# Autodesk Inventor assembly: 000-A-000
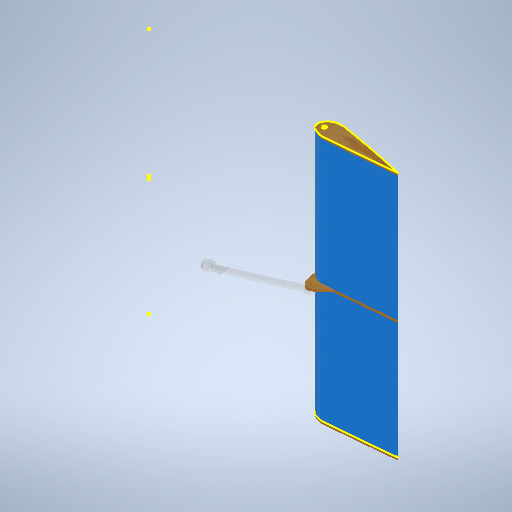
[picture p0: Inventor's stored thumbnail of the model, 512x512]
Saved by Autodesk Inventor 2025.1 (Build 291241000, 241)
## iProperties
Created: 2025-01-30
Part Number: 000-A-000
Document SubType Name: Assembly
Designer: Carriett 4
Category: <PROJECT CATAGORY>
Title: <TITLE>
Author: Carriett 4
Revision Number: A
## Documents named in this file (14)
- C:\Users\chowg\OneDrive\Documents\Inventor\AVDASI 2 Group Project\assembly\4A.01.02.06-BC-v1-Final Aileron Assembly 80deg.iam
- C:\Users\chowg\OneDrive\Documents\Inventor\AVDASI 2 Group Project\assembly\4P.01.02.20-BC-v1-Middle Connecting Rib.ipt
- C:\Users\chowg\OneDrive\Documents\Inventor\AVDASI 2 Group Project\assembly\4P.01.02.21-BC-v1-Inboard Foam Rib.ipt
- C:\Users\chowg\OneDrive\Documents\Inventor\AVDASI 2 Group Project\assembly\4P.01.02.22-BC-v1-Outboard Foam Rib.ipt
- C:\Users\chowg\OneDrive\Documents\Inventor\AVDASI 2 Group Project\assembly\4P.01.02.27-BC-v1-Final Aileron L2 80deg.ipt
- C:\Users\chowg\OneDrive\Documents\Inventor\AVDASI 2 Group Project\assembly\4P.01.02.28-BC-v1-Final Aileron L3 80deg.ipt
- C:\Users\chowg\OneDrive\Documents\Inventor\AVDASI 2 Group Project\assembly\4P.01.02.17-BC-v1-End Rib.ipt
- C:\Users\Carriett 4\OneDrive\CAD library\AILERON ASSEMBLY\FinalAssemblyAileron290125\4P.01.02.20-BC-v1-Middle Connecting Rib.ipt
- C:\Users\Carriett 4\OneDrive\CAD library\AILERON ASSEMBLY\FinalAssemblyAileron290125\4P.01.02.21-BC-v1-Inboard Foam Rib.ipt
- C:\Users\Carriett 4\OneDrive\CAD library\AILERON ASSEMBLY\FinalAssemblyAileron290125\4P.01.02.22-BC-v1-Outboard Foam Rib.ipt
- C:\Users\Carriett 4\OneDrive\CAD library\AILERON ASSEMBLY\FinalAssemblyAileron290125\4P.01.02.27-BC-v1-Final Aileron L2 80deg.ipt
- C:\Users\Carriett 4\OneDrive\CAD library\AILERON ASSEMBLY\FinalAssemblyAileron290125\4P.01.02.28-BC-v1-Final Aileron L3 80deg.ipt
- C:\Users\Carriett 4\OneDrive\CAD library\AILERON ASSEMBLY\FinalAssemblyAileron290125\4P.01.02.17-BC-v1-End Rib.ipt
- C:\Users\me19654\OneDrive - University of Bristol\PhD Project\005 Design (CAD and schematics)\001 Wind Tunnel\CAD Library\001-A-017 CONTRACTION ASSY.iam
## Components (7 placed, 6 different names)
1. 4P.01.02.20-BC-v1-Middle Connecting Rib:1 — Rigid:2, Rigid:3, Rotational:1, Rigid:4, Rigid:6
2. 4P.01.02.21-BC-v1-Inboard Foam Rib:1 — Rigid:2, Mate:1, Rigid:4
3. 4P.01.02.22-BC-v1-Outboard Foam Rib:1 — Rigid:3, Rigid:5, Rigid:6
4. 4P.01.02.27-BC-v1-Final Aileron L2 80deg:1 — Rotational:2
5. 4P.01.02.28-BC-v1-Final Aileron L3 80deg:1 — Rotational:1, Rotational:2
6. 4P.01.02.17-BC-v1-End Rib:1 — Mate:1
7. 4P.01.02.17-BC-v1-End Rib:2 — Rigid:5
## Relationships (8: WeldJoint 5, RevoluteJoint 2, Mate 1)
- Rigid:2 [WeldJoint]: 4P.01.02.20-BC-v1-Middle Connecting Rib:1 ↔ 4P.01.02.21-BC-v1-Inboard Foam Rib:1
- Rigid:3 [WeldJoint]: 4P.01.02.20-BC-v1-Middle Connecting Rib:1 ↔ 4P.01.02.22-BC-v1-Outboard Foam Rib:1
- Rotational:1 [RevoluteJoint]: 4P.01.02.20-BC-v1-Middle Connecting Rib:1 ↔ 4P.01.02.28-BC-v1-Final Aileron L3 80deg:1
- Rotational:2 [RevoluteJoint]: 4P.01.02.27-BC-v1-Final Aileron L2 80deg:1 ↔ 4P.01.02.28-BC-v1-Final Aileron L3 80deg:1
- Mate:1: 4P.01.02.21-BC-v1-Inboard Foam Rib:1 ↔ 4P.01.02.17-BC-v1-End Rib:1
- Rigid:4 [WeldJoint]: 4P.01.02.20-BC-v1-Middle Connecting Rib:1 ↔ 4P.01.02.21-BC-v1-Inboard Foam Rib:1
- Rigid:5 [WeldJoint]: 4P.01.02.22-BC-v1-Outboard Foam Rib:1 ↔ 4P.01.02.17-BC-v1-End Rib:2
- Rigid:6 [WeldJoint]: 4P.01.02.20-BC-v1-Middle Connecting Rib:1 ↔ 4P.01.02.22-BC-v1-Outboard Foam Rib:1
